# Autodesk Inventor assembly: stand
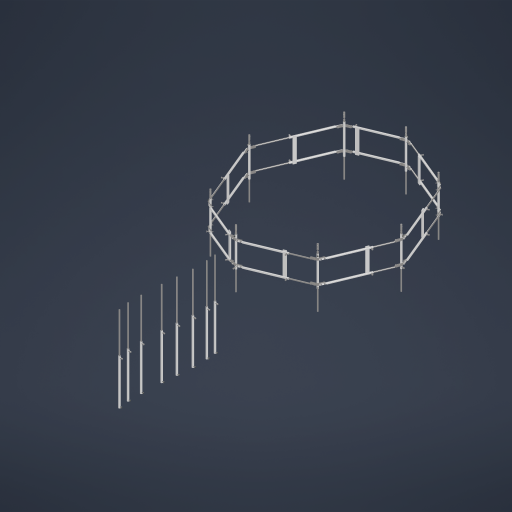
[picture p0: Inventor's stored thumbnail of the model, 512x512]
Saved by Autodesk Inventor 2023 (Build 270158000, 158)
## iProperties
Created: 2022-04-27
Part Number: stand
Document SubType Name: Assembly
Designer: Norbert Ligas
Author: Norbert Ligas
## Documents named in this file (4)
- C:\Users\norbe\Repozytoria\NormalMapScanner\stand_construction\stand.iam
- C:\Users\norbe\Repozytoria\NormalMapScanner\stand_construction\parts\adjustable_leg.iam
- C:\Users\norbe\Repozytoria\NormalMapScanner\stand_construction\parts\adjustable_double_connector.iam
- C:\Users\norbe\Repozytoria\NormalMapScanner\stand_construction\parts\adjustable_arm.iam
## Components (24 placed, 3 different names)
1. adjustable_leg:1 [sub-assembly] — Mate:1, Flush:1, Flush:2, Flush:3, Tangent:1, Mate:4, Mate:6, Mate:7, Mate:8, Mate:67, Mate:68, Mate:69, Mate:70, Tangent:30, Tangent:31
2. adjustable_leg:2 [sub-assembly] — Mate:10, Mate:11, Mate:12, Flush:14, Tangent:3, Mate:13, Mate:14, Mate:15, Mate:16, Mate:17, Tangent:4, Tangent:5
3. adjustable_leg:3 [sub-assembly] — Tangent:6, Mate:18, Mate:19, Mate:20, Mate:21, Tangent:7, Tangent:8, Mate:22, Mate:23, Mate:24, Mate:25, Tangent:9, Mate:71
4. adjustable_leg:4 [sub-assembly] — Tangent:10, Mate:26, Mate:27, Mate:28, Mate:29, Tangent:11, Mate:30, Tangent:12, Mate:31, Mate:32, Mate:33, Tangent:13, Mate:72
5. adjustable_leg:5 [sub-assembly] — Tangent:14, Mate:34, Mate:35, Mate:36, Mate:37, Tangent:15, Mate:39, Tangent:16, Tangent:17, Mate:40, Mate:41, Mate:42, Mate:73
6. adjustable_leg:6 [sub-assembly] — Mate:43, Mate:44, Mate:45, Mate:46, Tangent:18, Tangent:19, Mate:47, Mate:48, Mate:49, Mate:50, Tangent:20, Tangent:21, Mate:74
7. adjustable_leg:7 [sub-assembly] — Mate:51, Mate:52, Mate:53, Mate:54, Tangent:22, Tangent:23, Mate:55, Mate:56, Mate:57, Mate:58, Tangent:24, Tangent:25, Mate:75
8. adjustable_leg:8 [sub-assembly] — Mate:59, Mate:60, Mate:61, Mate:62, Tangent:26, Tangent:27, Mate:63, Mate:64, Mate:65, Mate:66, Tangent:28, Tangent:29, Mate:76
9. adjustable_double_connector:1 [sub-assembly] — Mate:14, Mate:15, Mate:16, Mate:17, Tangent:4, Tangent:5, Tangent:6, Mate:18, Mate:19, Mate:20, Mate:21, Tangent:7
10. adjustable_double_connector:2 [sub-assembly] — Tangent:8, Mate:22, Mate:23, Mate:24, Mate:25, Tangent:9, Tangent:10, Mate:26, Mate:27, Mate:28, Mate:29, Tangent:11
11. adjustable_double_connector:3 [sub-assembly] — Mate:30, Tangent:12, Mate:31, Mate:32, Mate:33, Tangent:13, Tangent:14, Mate:34, Mate:35, Mate:36, Mate:37, Tangent:15
12. adjustable_double_connector:4 [sub-assembly] — Mate:39, Tangent:16, Tangent:17, Mate:40, Mate:41, Mate:42, Mate:43, Mate:44, Mate:45, Mate:46, Tangent:18, Tangent:19
13. adjustable_double_connector:5 [sub-assembly] — Mate:47, Mate:48, Mate:49, Mate:50, Tangent:20, Tangent:21, Mate:51, Mate:52, Mate:53, Mate:54, Tangent:22, Tangent:23
14. adjustable_double_connector:6 [sub-assembly] — Mate:55, Mate:56, Mate:57, Mate:58, Tangent:24, Tangent:25, Mate:59, Mate:60, Mate:61, Mate:62, Tangent:26, Tangent:27
15. adjustable_double_connector:7 [sub-assembly] — Mate:63, Mate:64, Mate:65, Mate:66, Tangent:28, Tangent:29, Mate:67, Mate:68, Mate:69, Mate:70, Tangent:30, Tangent:31
16. adjustable_double_connector:8 [sub-assembly] — Tangent:1, Mate:4, Mate:6, Mate:7, Mate:8, Mate:10, Mate:11, Mate:12, Angle:1, Tangent:2, Tangent:3, Mate:13
17. adjustable_arm:1 [sub-assembly]
18. adjustable_arm:2 [sub-assembly]
19. adjustable_arm:3 [sub-assembly]
20. adjustable_arm:4 [sub-assembly]
21. adjustable_arm:5 [sub-assembly]
22. adjustable_arm:6 [sub-assembly]
23. adjustable_arm:7 [sub-assembly]
24. adjustable_arm:8 [sub-assembly]
## Relationships (107: Mate 71, Tangent 31, Flush 4, Angle 1)
- Mate:1: adjustable_leg:1
- Flush:1: adjustable_leg:1
- Flush:2: adjustable_leg:1
- Flush:3: adjustable_leg:1
- Tangent:1: adjustable_leg:1 ↔ adjustable_double_connector:8
- Mate:4: adjustable_leg:1 ↔ adjustable_double_connector:8
- Mate:6: adjustable_leg:1 ↔ adjustable_double_connector:8
- Mate:7: adjustable_leg:1 ↔ adjustable_double_connector:8
- Mate:8: adjustable_leg:1 ↔ adjustable_double_connector:8
- Mate:10: adjustable_leg:2 ↔ adjustable_double_connector:8
- Mate:11: adjustable_leg:2 ↔ adjustable_double_connector:8
- Mate:12: adjustable_leg:2 ↔ adjustable_double_connector:8
- Flush:14: adjustable_leg:2
- Angle:1 (0 deg): adjustable_double_connector:8
- Tangent:2: adjustable_double_connector:8
- Tangent:3: adjustable_leg:2 ↔ adjustable_double_connector:8
- Mate:13: adjustable_leg:2 ↔ adjustable_double_connector:8
- Mate:14: adjustable_leg:2 ↔ adjustable_double_connector:1
- Mate:15: adjustable_leg:2 ↔ adjustable_double_connector:1
- Mate:16: adjustable_leg:2 ↔ adjustable_double_connector:1
- Mate:17: adjustable_leg:2 ↔ adjustable_double_connector:1
- Tangent:4: adjustable_leg:2 ↔ adjustable_double_connector:1
- Tangent:5: adjustable_leg:2 ↔ adjustable_double_connector:1
- Tangent:6: adjustable_leg:3 ↔ adjustable_double_connector:1
- Mate:18: adjustable_leg:3 ↔ adjustable_double_connector:1
- Mate:19: adjustable_leg:3 ↔ adjustable_double_connector:1
- Mate:20: adjustable_leg:3 ↔ adjustable_double_connector:1
- Mate:21: adjustable_leg:3 ↔ adjustable_double_connector:1
- Tangent:7: adjustable_leg:3 ↔ adjustable_double_connector:1
- Tangent:8: adjustable_leg:3 ↔ adjustable_double_connector:2
- Mate:22: adjustable_leg:3 ↔ adjustable_double_connector:2
- Mate:23: adjustable_leg:3 ↔ adjustable_double_connector:2
- Mate:24: adjustable_leg:3 ↔ adjustable_double_connector:2
- Mate:25: adjustable_leg:3 ↔ adjustable_double_connector:2
- Tangent:9: adjustable_leg:3 ↔ adjustable_double_connector:2
- Tangent:10: adjustable_leg:4 ↔ adjustable_double_connector:2
- Mate:26: adjustable_leg:4 ↔ adjustable_double_connector:2
- Mate:27: adjustable_leg:4 ↔ adjustable_double_connector:2
- Mate:28: adjustable_leg:4 ↔ adjustable_double_connector:2
- Mate:29: adjustable_leg:4 ↔ adjustable_double_connector:2
- Tangent:11: adjustable_leg:4 ↔ adjustable_double_connector:2
- Mate:30: adjustable_leg:4 ↔ adjustable_double_connector:3
- Tangent:12: adjustable_leg:4 ↔ adjustable_double_connector:3
- Mate:31: adjustable_leg:4 ↔ adjustable_double_connector:3
- Mate:32: adjustable_leg:4 ↔ adjustable_double_connector:3
- Mate:33: adjustable_leg:4 ↔ adjustable_double_connector:3
- Tangent:13: adjustable_leg:4 ↔ adjustable_double_connector:3
- Tangent:14: adjustable_leg:5 ↔ adjustable_double_connector:3
- Mate:34: adjustable_leg:5 ↔ adjustable_double_connector:3
- Mate:35: adjustable_leg:5 ↔ adjustable_double_connector:3
- Mate:36: adjustable_leg:5 ↔ adjustable_double_connector:3
- Mate:37: adjustable_leg:5 ↔ adjustable_double_connector:3
- Tangent:15: adjustable_leg:5 ↔ adjustable_double_connector:3
- Mate:39: adjustable_leg:5 ↔ adjustable_double_connector:4
- Tangent:16: adjustable_leg:5 ↔ adjustable_double_connector:4
- Tangent:17: adjustable_leg:5 ↔ adjustable_double_connector:4
- Mate:40: adjustable_leg:5 ↔ adjustable_double_connector:4
- Mate:41: adjustable_leg:5 ↔ adjustable_double_connector:4
- Mate:42: adjustable_leg:5 ↔ adjustable_double_connector:4
- Mate:43: adjustable_leg:6 ↔ adjustable_double_connector:4
- Mate:44: adjustable_leg:6 ↔ adjustable_double_connector:4
- Mate:45: adjustable_leg:6 ↔ adjustable_double_connector:4
- Mate:46: adjustable_leg:6 ↔ adjustable_double_connector:4
- Tangent:18: adjustable_leg:6 ↔ adjustable_double_connector:4
- Tangent:19: adjustable_leg:6 ↔ adjustable_double_connector:4
- Mate:47: adjustable_leg:6 ↔ adjustable_double_connector:5
- Mate:48: adjustable_leg:6 ↔ adjustable_double_connector:5
- Mate:49: adjustable_leg:6 ↔ adjustable_double_connector:5
- Mate:50: adjustable_leg:6 ↔ adjustable_double_connector:5
- Tangent:20: adjustable_leg:6 ↔ adjustable_double_connector:5
- Tangent:21: adjustable_leg:6 ↔ adjustable_double_connector:5
- Mate:51: adjustable_leg:7 ↔ adjustable_double_connector:5
- Mate:52: adjustable_leg:7 ↔ adjustable_double_connector:5
- Mate:53: adjustable_leg:7 ↔ adjustable_double_connector:5
- Mate:54: adjustable_leg:7 ↔ adjustable_double_connector:5
- Tangent:22: adjustable_leg:7 ↔ adjustable_double_connector:5
- Tangent:23: adjustable_leg:7 ↔ adjustable_double_connector:5
- Mate:55: adjustable_leg:7 ↔ adjustable_double_connector:6
- Mate:56: adjustable_leg:7 ↔ adjustable_double_connector:6
- Mate:57: adjustable_leg:7 ↔ adjustable_double_connector:6
- Mate:58: adjustable_leg:7 ↔ adjustable_double_connector:6
- Tangent:24: adjustable_leg:7 ↔ adjustable_double_connector:6
- Tangent:25: adjustable_leg:7 ↔ adjustable_double_connector:6
- Mate:59: adjustable_leg:8 ↔ adjustable_double_connector:6
- Mate:60: adjustable_leg:8 ↔ adjustable_double_connector:6
- Mate:61: adjustable_leg:8 ↔ adjustable_double_connector:6
- Mate:62: adjustable_leg:8 ↔ adjustable_double_connector:6
- Tangent:26: adjustable_leg:8 ↔ adjustable_double_connector:6
- Tangent:27: adjustable_leg:8 ↔ adjustable_double_connector:6
- Mate:63: adjustable_leg:8 ↔ adjustable_double_connector:7
- Mate:64: adjustable_leg:8 ↔ adjustable_double_connector:7
- Mate:65: adjustable_leg:8 ↔ adjustable_double_connector:7
- Mate:66: adjustable_leg:8 ↔ adjustable_double_connector:7
- Tangent:28: adjustable_leg:8 ↔ adjustable_double_connector:7
- Tangent:29: adjustable_leg:8 ↔ adjustable_double_connector:7
- Mate:67: adjustable_leg:1 ↔ adjustable_double_connector:7
- Mate:68: adjustable_leg:1 ↔ adjustable_double_connector:7
- Mate:69: adjustable_leg:1 ↔ adjustable_double_connector:7
- Mate:70: adjustable_leg:1 ↔ adjustable_double_connector:7
- Tangent:30: adjustable_leg:1 ↔ adjustable_double_connector:7
- Tangent:31: adjustable_leg:1 ↔ adjustable_double_connector:7
- Mate:71: adjustable_leg:3
- Mate:72: adjustable_leg:4
- Mate:73: adjustable_leg:5
- Mate:74: adjustable_leg:6
- Mate:75: adjustable_leg:7
- Mate:76: adjustable_leg:8
## Named parameters: arm_min_length = 300 mm, arm_max_length = 565 mm, max_extrusion = 265 mm, min_extrusion = 0 mm, hinge_insertion = 15 mm, connection_length = 20 mm, bar_length = 285 mm, pipe_length = 300 mm
